# Autodesk Inventor assembly: PivotMech
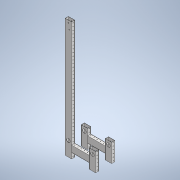
[picture p0: Inventor's stored thumbnail of the model, 180x180]
Saved by Autodesk Inventor 2022 (Build 260153000, 153)
## iProperties
Created: 2022-03-02
Part Number: PivotMech
Document SubType Name: Assembly
Designer: tagaz
Author: tagaz
## Documents named in this file (4)
- C:\Users\tagaz\OneDrive\Documents\T3-Cad\CAD\2022 Parts\TelescopeElev\PivotMech\PivotMech.iam
- C:\Users\tagaz\OneDrive\Documents\T3-Cad\CAD\2022 Parts\TelescopeElev\PivotMech\ElevatorPivotBar1.ipt
- C:\Users\tagaz\OneDrive\Documents\T3-Cad\CAD\2022 Parts\TelescopeElev\PivotMech\ElevatorPivotBar2.ipt
- C:\Users\tagaz\OneDrive\Documents\T3-Cad\CAD\2022 Parts\TelescopeElev\PivotMech\ElevatorPivotBar3.ipt
## Components (6 placed, 3 different names)
1. ElevatorPivotBar1:1 — Flush:1, Flush:2, Flush:3, Flush:4, Mate:6
2. ElevatorPivotBar3:2 — Flush:1, Flush:2, Flush:9, Mate:5, Flush:10, Mate:7
3. ElevatorPivotBar2:1 — Flush:3, Flush:4, Mate:6, Mate:7
4. ElevatorPivotBar1:3 — Mate:8
5. ElevatorPivotBar1:4 — Flush:9, Mate:5, Flush:10, Mate:9
6. ElevatorPivotBar2:2 — Mate:8, Mate:9
## Relationships (15: Flush 10, Mate 5)
- Flush:1: ElevatorPivotBar1:1 ↔ ElevatorPivotBar3:2
- Flush:2: ElevatorPivotBar1:1 ↔ ElevatorPivotBar3:2
- Flush:3: ElevatorPivotBar1:1 ↔ ElevatorPivotBar2:1
- Flush:4 (50.8 mm): ElevatorPivotBar1:1 ↔ ElevatorPivotBar2:1
- [Flush]: ElevatorPivotBar1:3 ↔ ElevatorPivotBar1:4
- [Flush]: ElevatorPivotBar1:3 ↔ ElevatorPivotBar1:4
- [Flush]: ElevatorPivotBar1:3 ↔ ElevatorPivotBar2:2
- [Flush] (50.8 mm): ElevatorPivotBar1:3 ↔ ElevatorPivotBar2:2
- Flush:9: ElevatorPivotBar3:2 ↔ ElevatorPivotBar1:4
- Mate:5 (101.6 mm): ElevatorPivotBar3:2 ↔ ElevatorPivotBar1:4
- Flush:10: ElevatorPivotBar3:2 ↔ ElevatorPivotBar1:4
- Mate:6: ElevatorPivotBar1:1 ↔ ElevatorPivotBar2:1
- Mate:7: ElevatorPivotBar3:2 ↔ ElevatorPivotBar2:1
- Mate:8: ElevatorPivotBar1:3 ↔ ElevatorPivotBar2:2
- Mate:9: ElevatorPivotBar1:4 ↔ ElevatorPivotBar2:2
## Named parameters: d6_d0 = 0 mm, d7_d1 = 0 mm, d8_d2 = 0 mm, d11_d5 = 50.8 mm
